# Autodesk Inventor assembly: Zahnstange
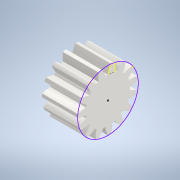
[picture p0: Inventor's stored thumbnail of the model, 180x180]
Saved by Autodesk Inventor 2021 (Build 250183000, 183)
## iProperties
Created: 2021-01-25
Part Number: Zahnstange
Document SubType Name: Assembly
Designer: Jaro Machnow
Author: Jaro Machnow
## Documents named in this file (3)
- C:\Users\Jaro Machnow\Documents\Vault\Gruppen\Gruppe 2\Entwurf\Amphibienfahrzeug\Wechsel zwischen Land und Wasser\Mechanik_zum_Wechseln\Zahnstange.iam
- C:\Users\Jaro Machnow\Documents\Vault\Gruppen\Gruppe 2\Entwurf\Amphibienfahrzeug\Wechsel zwischen Land und Wasser\Mechanik_zum_Wechseln\Zahnstange\Konstruktions-Assistent\Stirnräder3.iam
- C:\Users\Jaro Machnow\Documents\Vault\Gruppen\Gruppe 2\Entwurf\Amphibienfahrzeug\Wechsel zwischen Land und Wasser\Mechanik_zum_Wechseln\Zahnstange.ipt
## Components (2 placed, 2 different names)
1. Stirnräder:2 [sub-assembly] — Passend:1, Passend:2, Fluchtend:1
2. Zahnstange:1 — Fluchtend:1
## Relationships (3: Mate 2, Flush 1)
- Passend:1 [Mate]: Stirnräder:2
- Passend:2 [Mate]: Stirnräder:2
- Fluchtend:1 [Flush]: Stirnräder:2 ↔ Zahnstange:1
